# Autodesk Inventor assembly: side with gearbox
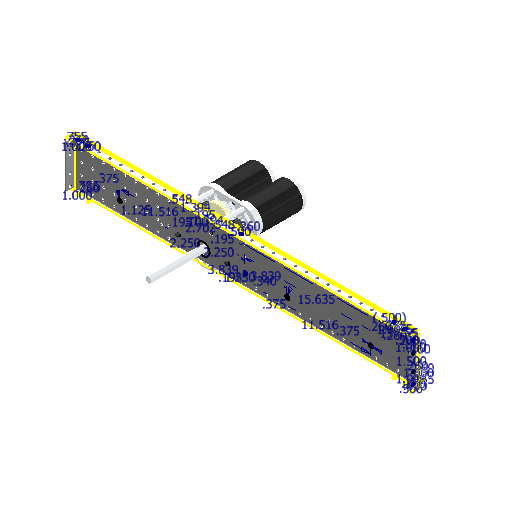
[picture p0: Inventor's stored thumbnail of the model, 512x512]
Saved by Autodesk Inventor 2022 (Build 260153000, 153)
## iProperties
Created: 2022-01-17
Part Number: side with gearbox
Document SubType Name: Assembly
Designer: 5126_Cad_2
Author: 5126_Cad_2
## Documents named in this file (4)
- A:\new 2022 cad\new 2022 cad\side with gearbox.iam
- A:\new 2022 cad\new 2022 cad\side pannel inner 2 00003.ipt
- side pannel 1 00001.ipt
- A:\new 2022 cad\new 2022 cad\WCP DS - Dual Speed Base Kit (217-3423).ipt
## Components (2 placed, 2 different names)
1. side pannel 1 00001:1 — Mate:1, Mate:2, Mate:3
2. WCP DS - Dual Speed Base Kit (217-3423):1 — Mate:1, Mate:2, Mate:3
## Relationships (3: Mate 3)
- Mate:1: side pannel 1 00001:1 ↔ WCP DS - Dual Speed Base Kit (217-3423):1
- Mate:2: side pannel 1 00001:1 ↔ WCP DS - Dual Speed Base Kit (217-3423):1
- Mate:3: side pannel 1 00001:1 ↔ WCP DS - Dual Speed Base Kit (217-3423):1
